# Autodesk Inventor assembly: spool 4 in
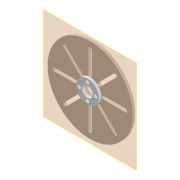
[picture p0: Inventor's stored thumbnail of the model, 180x180]
Saved by Autodesk Inventor 2020 (Build 240168000, 168)
## iProperties
Created: 2019-11-26
Part Number: spool 4 in
Document SubType Name: Assembly
Designer: ball
Author: ball
## Documents named in this file (3)
- C:\FTC\FTC8863CAD\2019 Robot\Delivery\spool 4 in.iam
- C:\FTC\FTC8863CAD\2019 Robot\Delivery\spool 4in outer plate.ipt
- C:\FTC\FTC8863CAD\2019 Robot\Delivery\spool 4in inner plate.ipt
## Components (2 placed, 2 different names)
1. spool 4in outer plate:1 — Flush:1, Flush:2
2. spool 4in inner plate:1 — Flush:1, Flush:2
## Relationships (2: Flush 2)
- Flush:1: spool 4in outer plate:1 ↔ spool 4in inner plate:1
- Flush:2: spool 4in outer plate:1 ↔ spool 4in inner plate:1
